# Autodesk Inventor assembly: SimuCarro
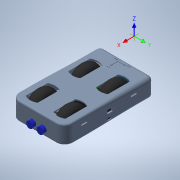
[picture p0: Inventor's stored thumbnail of the model, 180x180]
Saved by Autodesk Inventor 2021 (Build 250183000, 183)
## iProperties
Created: 2020-01-22
Part Number: SimuCarro
Document SubType Name: Assembly
Designer: peter
Author: peter
## Documents named in this file (13)
- C:\Users\peter\Documents\GitHub\Newton-Cart\3D Platform design\SimuCarro.iam
- C:\Users\peter\Documents\GitHub\Newton-Cart\3D Platform design\Barra.ipt
- C:\Users\peter\Documents\GitHub\Newton-Cart\3D Platform design\Bearing.ipt
- C:\Users\peter\Documents\GitHub\Newton-Cart\3D Platform design\Llanta.ipt
- C:\Users\peter\Documents\GitHub\Newton-Cart\3D Platform design\Carcasa1.ipt
- C:\Users\peter\Documents\GitHub\Newton-Cart\3D Platform design\Celda.ipt
- C:\Users\peter\Documents\GitHub\Newton-Cart\3D Platform design\garracomp2.ipt
- C:\Users\peter\Documents\GitHub\Newton-Cart\3D Platform design\Enc_.ipt
- C:\Users\peter\Documents\GitHub\Newton-Cart\3D Platform design\Carcasa2.ipt
- C:\Users\peter\Documents\GitHub\Newton-Cart\3D Platform design\Batt.ipt
- C:\Users\peter\Documents\GitHub\Newton-Cart\3D Platform design\PCB.ipt
- C:\Users\peter\Documents\GitHub\Newton-Cart\3D Platform design\HCSR04.ipt
- C:\Users\peter\Documents\GitHub\Newton-Cart\3D Platform design\HC020K.ipt
## Components (22 placed, 12 different names)
1. Barra:1 — Mate:30, Mate:31, Mate:46, Mate:55
2. Llanta:1 — Mate:30
3. Llanta:2 — Mate:31, Mate:46
4. Carcasa1:1 — Mate:20, Mate:25, Mate:26, Mate:27, Mate:28, Mate:32, Mate:33, Mate:40, Mate:41, Mate:42, Mate:43, Mate:45, Mate:48, Mate:50, Mate:51, Mate:53, Mate:54, Symmetry:1, Symmetry:3, Symmetry:4
5. Bearing:2 — Mate:21, Mate:22, Mate:28, Mate:54, Mate:55
6. Celda:1 — Mate:48, Mate:50, Mate:51
7. garracomp2:2 — Mate:20, Mate:21, Mate:22, Mate:26, Mate:33
8. garracomp2:3 — Mate:23, Mate:24, Mate:25, Mate:32
9. Bearing:3 — Mate:23, Mate:24, Mate:27, Mate:53
10. Barra:2 — Mate:44, Mate:45
11. Llanta:3
12. Llanta:4
13. Bearing:4 — Mate:41, Mate:44
14. garracomp2:4 — Mate:42
15. garracomp2:5 — Mate:43
16. Bearing:5 — Mate:40
17. Enc_:1
18. Carcasa2:1 — Symmetry:1, Symmetry:3
19. Batt:1
20. PCB:1
21. HCSR04:1 — Symmetry:4
22. HC020K:1
## Relationships (35: Mate 32, Symmetry 3)
- Mate:20: Carcasa1:1 ↔ garracomp2:2
- Mate:21: Bearing:2 ↔ garracomp2:2
- Mate:22: Bearing:2 ↔ garracomp2:2
- Mate:23: garracomp2:3 ↔ Bearing:3
- Mate:24: garracomp2:3 ↔ Bearing:3
- Mate:25: Carcasa1:1 ↔ garracomp2:3
- Mate:26: Carcasa1:1 ↔ garracomp2:2
- Mate:27: Carcasa1:1 ↔ Bearing:3
- Mate:28: Carcasa1:1 ↔ Bearing:2
- Mate:30: Barra:1 ↔ Llanta:1
- Mate:31: Barra:1 ↔ Llanta:2
- Mate:32: Carcasa1:1 ↔ garracomp2:3
- Mate:33: Carcasa1:1 ↔ garracomp2:2
- [Mate]: Bearing:4 ↔ garracomp2:4
- [Mate]: Bearing:4 ↔ garracomp2:4
- [Mate]: garracomp2:5 ↔ Bearing:5
- [Mate]: garracomp2:5 ↔ Bearing:5
- [Mate]: Barra:2 ↔ Llanta:3
- [Mate]: Barra:2 ↔ Llanta:4
- Mate:40: Carcasa1:1 ↔ Bearing:5
- Mate:41: Carcasa1:1 ↔ Bearing:4
- Mate:42: Carcasa1:1 ↔ garracomp2:4
- Mate:43: Carcasa1:1 ↔ garracomp2:5
- Mate:44: Barra:2 ↔ Bearing:4
- Mate:45: Carcasa1:1 ↔ Barra:2
- Mate:46: Barra:1 ↔ Llanta:2
- Mate:48: Carcasa1:1 ↔ Celda:1
- Mate:50: Carcasa1:1 ↔ Celda:1
- Mate:51: Carcasa1:1 ↔ Celda:1
- Mate:53: Carcasa1:1 ↔ Bearing:3
- Mate:54: Carcasa1:1 ↔ Bearing:2
- Mate:55: Barra:1 ↔ Bearing:2
- Symmetry:1: Carcasa1:1 ↔ Carcasa2:1
- Symmetry:3: Carcasa1:1 ↔ Carcasa2:1
- Symmetry:4: Carcasa1:1 ↔ HCSR04:1
## Named parameters: d47_d32 = 0 mm, d48_d33 = 0 mm, d49_d34 = 0 mm, d50_d35 = 0 mm, d51_d41 = 0 mm, d52_d42 = 0 mm
